# Autodesk Inventor assembly: okok last one
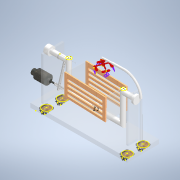
[picture p0: Inventor's stored thumbnail of the model, 180x180]
Saved by Autodesk Inventor 2022 (Build 260153000, 153)
## iProperties
Created: 2023-06-18
Part Number: okok last one
Document SubType Name: Assembly
Designer: Preeti Anand
Author: Preeti Anand
## Documents named in this file (14)
- C:\Users\jyoti\Downloads\okok last one.iam
- C:\Users\jyoti\Downloads\Cradlemotor.ipt
- C:\Users\jyoti\Downloads\LStand.ipt
- C:\Users\jyoti\Downloads\FinalAssembly.iam
- C:\Users\jyoti\Downloads\main toy.ipt
- C:\Users\jyoti\Downloads\new wheels.ipt
- C:\Users\jyoti\Downloads\5cmextender.ipt
- C:\Users\jyoti\Downloads\111toystand.ipt
- C:\Users\jyoti\Downloads\new 2nd extender.ipt
- C:\Users\jyoti\Downloads\newhands.ipt
- C:\Users\jyoti\Downloads\10cmlinks.ipt
- C:\Users\jyoti\OneDrive\Desktop\auto desk\new bigger lick 2 small.ipt
- C:\Users\jyoti\OneDrive\Desktop\auto desk\somme link.ipt
- C:\Users\jyoti\OneDrive\Desktop\auto desk\jointrod.ipt
## Components (16 placed, 13 different names)
1. Cradlemotor:2 — Mate:2, Mate:3, Mate:31, Mate:32
2. LStand:1 — Mate:2, Mate:3, Mate:24, Mate:25, Mate:26, Mate:27, Mate:29, Mate:40, Rotational:6
3. new wheels:2 — Mate:25
4. new wheels:3 — Mate:26
5. new wheels:4 — Mate:24
6. new wheels:5 — Mate:27
7. 5cmextender:1 — Rotational:2, Mate:28
8. 111toystand:1 — Rotational:2, Rotational:6
9. main toy:1 — Rotational:4
10. new 2nd extender:1 — Mate:28, Rotational:4
11. newhands:1 — Mate:29, Mate:30, Mate:39, Rotational:5, Mate:40
12. 10cmlinks:1 — Mate:33, Mate:34, Mate:35, Mate:36
13. new bigger lick 2 small:1 — Mate:31, Mate:32, Mate:33, Mate:34
14. somme link:1 — Mate:30, Mate:35, Mate:36, Mate:37, Mate:38
15. jointrod:1 — Mate:37, Mate:38, Mate:39
16. FinalAssembly:1 [sub-assembly] — Rotational:5
## Relationships (23: Mate 19, RevoluteJoint 4)
- Mate:2: Cradlemotor:2 ↔ LStand:1
- Mate:3: Cradlemotor:2 ↔ LStand:1
- Mate:24: LStand:1 ↔ new wheels:4
- Mate:25: LStand:1 ↔ new wheels:2
- Mate:26: LStand:1 ↔ new wheels:3
- Mate:27: LStand:1 ↔ new wheels:5
- Rotational:2 [RevoluteJoint]: 5cmextender:1 ↔ 111toystand:1
- Mate:28: 5cmextender:1 ↔ new 2nd extender:1
- Rotational:4 [RevoluteJoint]: main toy:1 ↔ new 2nd extender:1
- Mate:29: LStand:1 ↔ newhands:1
- Mate:30: newhands:1 ↔ somme link:1
- Mate:31: Cradlemotor:2 ↔ new bigger lick 2 small:1
- Mate:32: Cradlemotor:2 ↔ new bigger lick 2 small:1
- Mate:33: 10cmlinks:1 ↔ new bigger lick 2 small:1
- Mate:34: 10cmlinks:1 ↔ new bigger lick 2 small:1
- Mate:35: 10cmlinks:1 ↔ somme link:1
- Mate:36: 10cmlinks:1 ↔ somme link:1
- Mate:37: somme link:1 ↔ jointrod:1
- Mate:38: somme link:1 ↔ jointrod:1
- Mate:39: newhands:1 ↔ jointrod:1
- Rotational:5 [RevoluteJoint]: newhands:1 ↔ FinalAssembly:1
- Mate:40: LStand:1 ↔ newhands:1
- Rotational:6 [RevoluteJoint]: LStand:1 ↔ 111toystand:1
